# Autodesk Inventor assembly: HolderAssembly
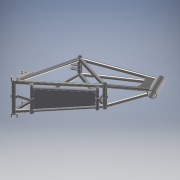
[picture p0: Inventor's stored thumbnail of the model, 180x180]
Saved by Autodesk Inventor 2019.3 (Build 233278000, 278)
## iProperties
Created: 2018-10-02
Part Number: HolderAssembly
Document SubType Name: Assembly
Designer: eroldan
Author: eroldan
## Documents named in this file (3)
- C:\Users\eroldan\Desktop\3dprojects\OpenEmoto\MainFrame\Battery\LowerCageJig\HolderAssembly.iam
- C:\Users\eroldan\Desktop\3dprojects\OpenEmoto\MainFrame\Battery\Assembly.iam
- C:\Users\eroldan\Desktop\3dprojects\OpenEmoto\MainFrame\Battery\LowerCageJig\Holders.ipt
## Components (2 placed, 2 different names)
1. Assembly:1 [sub-assembly]
2. Holders:1 — Flush:1
## Relationships (1: Flush 1)
- Flush:1: Holders:1
